# Autodesk Inventor assembly: weapon assembly
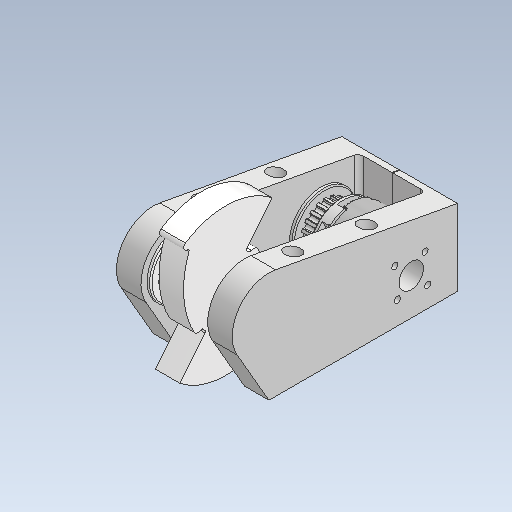
[picture p0: Inventor's stored thumbnail of the model, 512x512]
Saved by Autodesk Inventor 2026.4 (Build 304435030, 435C)
## iProperties
Created: 2026-11-20
Part Number: weapon assembly
Document SubType Name: Assembly
Designer: weira
Author: weira
## Documents named in this file (7)
- C:\Users\weira\OneDrive\Desktop\Battlebot Projekt\Battle-Bot-Project\Version2\weapon_assembly\weapon assembly.iam
- C:\Users\weira\OneDrive\Desktop\Battlebot Projekt\Battle-Bot-Project\Version2\weapon_assembly\Waffenhalterung  rechts.ipt
- C:\Users\weira\OneDrive\Desktop\Battlebot Projekt\Battle-Bot-Project\Version2\weapon_assembly\Waffenhalterung  links.ipt
- C:\Users\weira\OneDrive\Desktop\Battlebot Projekt\Battle-Bot-Project\Version2\Kaufteile\MT2204_Brushless_Motor.ipt
- C:\Users\weira\OneDrive\Desktop\Battlebot Projekt\Battle-Bot-Project\Version2\weapon_assembly\Riemenscheibe HTD_3M.ipt
- C:\Users\weira\OneDrive\Desktop\Battlebot Projekt\Battle-Bot-Project\Version2\weapon_assembly\Waffendesign_mit_Infilloptimierung.ipt
- C:\Users\weira\OneDrive\Desktop\Battlebot Projekt\Battle-Bot-Project\Version2\Kaufteile\Gewindemuffe m3x25.ipt
## Components (9 placed, 6 different names)
1. Waffenhalterung  rechts:1 — Passend:1, Fluchtend:1, Passend:2, Passend:5, Passend:6, Passend:7, Passend:17, Fluchtend:6, Passend:20, Fluchtend:8
2. Waffenhalterung  links:1 — Fluchtend:2, Passend:3, Passend:12, Passend:14, Passend:18, Fluchtend:5, Passend:19, Fluchtend:7
3. MT2204_Brushless_Motor:1 — Passend:5, Passend:6, Passend:7, Passend:8, Passend:9, Passend:10
4. Riemenscheibe HTD_3M:1 — Passend:8, Passend:9, Passend:10, Passend:13
5. Waffendesign_mit_Infilloptimierung:1 — Passend:12, Passend:13, Passend:14
6. Gewindemuffe m3x25:3 — Passend:17, Fluchtend:6
7. Gewindemuffe m3x25:4 — Passend:18, Fluchtend:5
8. Gewindemuffe m3x25:5 — Passend:19, Fluchtend:7
9. Gewindemuffe m3x25:6 — Passend:20, Fluchtend:8
## Relationships (22: Mate 16, Flush 6)
- Passend:1 [Mate]: Waffenhalterung  rechts:1
- Fluchtend:1 [Flush] (-55 mm): Waffenhalterung  rechts:1
- Passend:2 [Mate]: Waffenhalterung  rechts:1
- Fluchtend:2 [Flush] (-55 mm): Waffenhalterung  links:1
- Passend:3 [Mate]: Waffenhalterung  links:1
- Passend:5 [Mate]: Waffenhalterung  rechts:1 ↔ MT2204_Brushless_Motor:1
- Passend:6 [Mate]: Waffenhalterung  rechts:1 ↔ MT2204_Brushless_Motor:1
- Passend:7 [Mate]: Waffenhalterung  rechts:1 ↔ MT2204_Brushless_Motor:1
- Passend:8 [Mate]: MT2204_Brushless_Motor:1 ↔ Riemenscheibe HTD_3M:1
- Passend:9 [Mate]: MT2204_Brushless_Motor:1 ↔ Riemenscheibe HTD_3M:1
- Passend:10 [Mate]: MT2204_Brushless_Motor:1 ↔ Riemenscheibe HTD_3M:1
- Passend:12 [Mate]: Waffenhalterung  links:1 ↔ Waffendesign_mit_Infilloptimierung:1
- Passend:13 [Mate]: Riemenscheibe HTD_3M:1 ↔ Waffendesign_mit_Infilloptimierung:1
- Passend:14 [Mate] (0.5 mm): Waffenhalterung  links:1 ↔ Waffendesign_mit_Infilloptimierung:1
- Passend:17 [Mate]: Waffenhalterung  rechts:1 ↔ Gewindemuffe m3x25:3
- Passend:18 [Mate]: Waffenhalterung  links:1 ↔ Gewindemuffe m3x25:4
- Fluchtend:5 [Flush]: Waffenhalterung  links:1 ↔ Gewindemuffe m3x25:4
- Fluchtend:6 [Flush]: Waffenhalterung  rechts:1 ↔ Gewindemuffe m3x25:3
- Passend:19 [Mate]: Waffenhalterung  links:1 ↔ Gewindemuffe m3x25:5
- Passend:20 [Mate]: Waffenhalterung  rechts:1 ↔ Gewindemuffe m3x25:6
- Fluchtend:7 [Flush]: Waffenhalterung  links:1 ↔ Gewindemuffe m3x25:5
- Fluchtend:8 [Flush]: Waffenhalterung  rechts:1 ↔ Gewindemuffe m3x25:6
